# Autodesk Inventor assembly: Motor
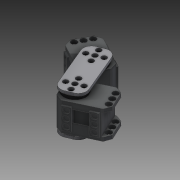
[picture p0: Inventor's stored thumbnail of the model, 180x180]
Saved by Autodesk Inventor 2014 (Build 180170000, 170)
## iProperties
Created: 2014-03-07
Part Number: Motor
Document SubType Name: Assembly
Designer: Grégoire
Author: Grégoire
## Documents named in this file (5)
- C:\Users\Bless\Desktop\XL320\src\Motor.iam
- C:\Users\Bless\Desktop\XL320\src\Motor.ipt
- C:\Users\Bless\Desktop\XL320\src\Arm.ipt
- C:\Users\Bless\Desktop\XL320\src\CounterArm.ipt
- C:\Users\Bless\Desktop\XL320\src\ArmToArm.ipt
## Components (8 placed, 4 different names)
1. Motor:1 — Placage:1, Placage:2, Placage:3, Placage:4
2. Arm:1 — Placage:3, Placage:4, Placage:9, Placage:13, Placage:14
3. CounterArm:1 — Placage:1, Placage:2, Placage:10, Placage:11, Placage:12
4. Motor:2 — Placage:17
5. Arm:2 — Placage:16, Placage:18
6. CounterArm:2 — Placage:15, Placage:19, Placage:20
7. ArmToArm:1 — Placage:10, Placage:11, Placage:12, Placage:15, Placage:19, Placage:20
8. ArmToArm:2 — Placage:9, Placage:13, Placage:14, Placage:16, Placage:17, Placage:18
## Relationships (20: Mate 20)
- Placage:1 [Mate]: Motor:1 ↔ CounterArm:1
- Placage:2 [Mate]: Motor:1 ↔ CounterArm:1
- Placage:3 [Mate]: Motor:1 ↔ Arm:1
- Placage:4 [Mate]: Motor:1 ↔ Arm:1
- [Mate]: Motor:2 ↔ CounterArm:2
- [Mate]: Motor:2 ↔ CounterArm:2
- [Mate]: Motor:2 ↔ Arm:2
- [Mate]: Motor:2 ↔ Arm:2
- Placage:9 [Mate]: Arm:1 ↔ ArmToArm:2
- Placage:10 [Mate]: CounterArm:1 ↔ ArmToArm:1
- Placage:11 [Mate]: CounterArm:1 ↔ ArmToArm:1
- Placage:12 [Mate]: CounterArm:1 ↔ ArmToArm:1
- Placage:13 [Mate]: Arm:1 ↔ ArmToArm:2
- Placage:14 [Mate]: Arm:1 ↔ ArmToArm:2
- Placage:15 [Mate]: CounterArm:2 ↔ ArmToArm:1
- Placage:16 [Mate]: Arm:2 ↔ ArmToArm:2
- Placage:17 [Mate]: Motor:2 ↔ ArmToArm:2
- Placage:18 [Mate]: Arm:2 ↔ ArmToArm:2
- Placage:19 [Mate]: CounterArm:2 ↔ ArmToArm:1
- Placage:20 [Mate]: CounterArm:2 ↔ ArmToArm:1
## Named parameters: d4_d0 = 0 mm, d5_d1 = 0 mm, d6_d2 = 0 mm, d7_d3 = 0 mm
